# Autodesk Inventor assembly: 000 ASY GBK Gubkinskiy
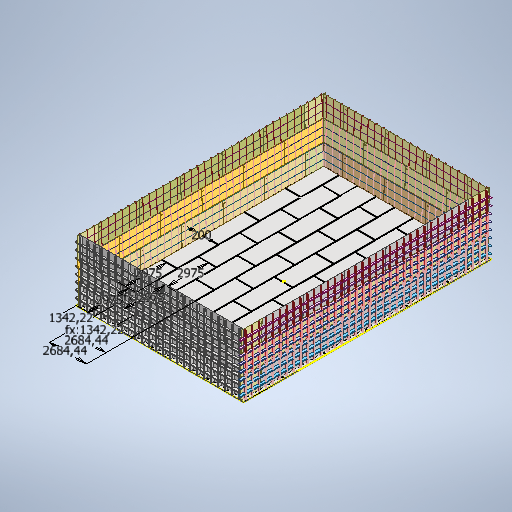
[picture p0: Inventor's stored thumbnail of the model, 512x512]
Saved by Autodesk Inventor 2026 (Build 300175000, 175)
## iProperties
Created: 2026-04-17
Part Number: 000 ASY GBK Gubkinskiy
Document SubType Name: Assembly
Designer: admin
Mass: 2.02017e+07 g
Surface Area: 1.30705e+07 cm^2
Volume: 2.57346e+06 cm^3
Density: 7.85 g/cm^3
Author: admin
## Documents named in this file (11)
- C:\Users\pokla\Documents\Inventor\GBK-Gubkinskiy\000 ASY GBK Gubkinskiy.iam
- C:\Users\pokla\Documents\Inventor\GBK-Gubkinskiy\GBK bottom.ipt
- C:\Users\pokla\Documents\Inventor\GBK-Gubkinskiy\GBK dummy wall 1.ipt
- C:\Users\pokla\Documents\Inventor\GBK-Gubkinskiy\GBK dummy wall 4.ipt
- C:\Users\pokla\Documents\Inventor\GBK-Gubkinskiy\GBK overall model.ipt
- C:\Users\pokla\Documents\Inventor\GBK-Gubkinskiy\ASY GBK 3110 wall shield Center 1.iam
- C:\Users\pokla\Documents\Inventor\GBK-Gubkinskiy\ASY GBK 3210 wall shield Center 3.iam
- C:\Users\pokla\Documents\Inventor\GBK-Gubkinskiy\ASY GBK 3310 wall shield Center 4.iam
- C:\Users\pokla\Documents\Inventor\GBK-Gubkinskiy\ASY GBK длинная стенка.iam
- C:\Users\pokla\Documents\Inventor\GBK-Gubkinskiy\090 ASY bottom.iam
- C:\Users\pokla\Documents\Inventor\GBK-Gubkinskiy\ASY GBK короткая стенка.iam
## Components (13 placed, 11 different names)
1. GBK bottom.ipt:1 — Совмещение:10, Совмещение:11, Совмещение:12, Совмещение:13, Совмещение:14, Жесткий:1, Заподлицо:7, Заподлицо:8, Заподлицо:9, Заподлицо:13, Совмещение:20, Совмещение:21, Заподлицо:14, Заподлицо:15, Совмещение:22, Заподлицо:16
2. GBK dummy wall 1.ipt:1 — Совмещение:10
3. GBK dummy wall 1.ipt:2 — Совмещение:11, Совмещение:12
4. GBK dummy wall 4.ipt:1 — Совмещение:13, Совмещение:14
5. GBK overall model.ipt:1 — Жесткий:1
6. ASY GBK длинная стенка.iam:1 [sub-assembly] — Заподлицо:15, Заподлицо:17
7. ASY GBK длинная стенка.iam:2 [sub-assembly] — Заподлицо:9, Заподлицо:12, Совмещение:21, Заподлицо:14
8. ASY GBK 3210 wall shield Center 3.iam:1 [sub-assembly] — Жесткий:2, Жесткий:3
9. ASY GBK 3310 wall shield Center 4.iam:1 [sub-assembly] — Жесткий:3
10. ASY GBK 3110 wall shield Center 1.iam:1 [sub-assembly] — Жесткий:2, Совмещение:18, Заподлицо:7
11. 090 ASY bottom.iam:1 [sub-assembly] — Совмещение:19, Заподлицо:8
12. ASY GBK короткая стенка.iam:1 [sub-assembly] — Заподлицо:12, Заподлицо:13, Совмещение:20
13. ASY GBK короткая стенка:2 [sub-assembly] — Совмещение:22, Заподлицо:16, Заподлицо:17
## Relationships (24: Mate 11, Flush 10, WeldJoint 3)
- [Flush]: GBK bottom.ipt:1 ↔ ASY GBK длинная стенка.iam:1
- [Mate]: GBK bottom.ipt:1 ↔ ASY GBK длинная стенка.iam:1
- Совмещение:10 [Mate]: GBK bottom.ipt:1 ↔ GBK dummy wall 1.ipt:1
- Совмещение:11 [Mate]: GBK bottom.ipt:1 ↔ GBK dummy wall 1.ipt:2
- Совмещение:12 [Mate]: GBK bottom.ipt:1 ↔ GBK dummy wall 1.ipt:2
- Совмещение:13 [Mate]: GBK bottom.ipt:1 ↔ GBK dummy wall 4.ipt:1
- Совмещение:14 [Mate]: GBK bottom.ipt:1 ↔ GBK dummy wall 4.ipt:1
- Жесткий:1 [WeldJoint]: GBK bottom.ipt:1 ↔ GBK overall model.ipt:1
- Жесткий:2 [WeldJoint]: ASY GBK 3210 wall shield Center 3.iam:1 ↔ ASY GBK 3110 wall shield Center 1.iam:1
- Жесткий:3 [WeldJoint]: ASY GBK 3210 wall shield Center 3.iam:1 ↔ ASY GBK 3310 wall shield Center 4.iam:1
- Совмещение:18 [Mate]: ASY GBK 3110 wall shield Center 1.iam:1
- Заподлицо:7 [Flush]: GBK bottom.ipt:1 ↔ ASY GBK 3110 wall shield Center 1.iam:1
- Совмещение:19 [Mate]: 090 ASY bottom.iam:1
- Заподлицо:8 [Flush]: GBK bottom.ipt:1 ↔ 090 ASY bottom.iam:1
- Заподлицо:9 [Flush]: GBK bottom.ipt:1 ↔ ASY GBK длинная стенка.iam:2
- Заподлицо:12 [Flush] (235 mm): ASY GBK длинная стенка.iam:2 ↔ ASY GBK короткая стенка.iam:1
- Заподлицо:13 [Flush] (20 mm): GBK bottom.ipt:1 ↔ ASY GBK короткая стенка.iam:1
- Совмещение:20 [Mate]: GBK bottom.ipt:1 ↔ ASY GBK короткая стенка.iam:1
- Совмещение:21 [Mate]: GBK bottom.ipt:1 ↔ ASY GBK длинная стенка.iam:2
- Заподлицо:14 [Flush] (20 mm): GBK bottom.ipt:1 ↔ ASY GBK длинная стенка.iam:2
- Заподлицо:15 [Flush] (20 mm): GBK bottom.ipt:1 ↔ ASY GBK длинная стенка.iam:1
- Совмещение:22 [Mate]: GBK bottom.ipt:1 ↔ ASY GBK короткая стенка:2
- Заподлицо:16 [Flush] (20 mm): GBK bottom.ipt:1 ↔ ASY GBK короткая стенка:2
- Заподлицо:17 [Flush] (235 mm): ASY GBK длинная стенка.iam:1 ↔ ASY GBK короткая стенка:2
## Named parameters: Зазор_по_горизонту = 1 mm, d120_Зазор_по_горизонту = 1 mm, d141_Зазор_по_горизонту = 1 mm, d159_d141_Зазор_по_горизонту = 1 mm, d175_d141_Зазор_по_горизонту = 1 mm
